# Autodesk Inventor assembly: 276-2194.html
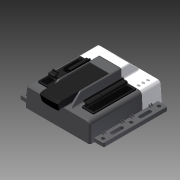
[picture p0: Inventor's stored thumbnail of the model, 180x180]
Saved by Autodesk Inventor 2013 (Build 170138000, 138)
## iProperties
Category: Logic
Company: Autodesk Inc.
Created: 2012-04-09
Part Number: 276-2194.html
Document SubType Name: Assembly
Designer: Autodesk Inc.
Catalog Web Link: http://www.vexrobotics.com/products/accessories/logic/276-2194.html#
Vendor: VEX
Mass: 136.985 g
Surface Area: 1281.69 cm^2
Volume: 120.224 cm^3
Author: Autodesk Inc.
## Documents named in this file (12)
- C:\Data Folder\VEX 2012\VEX KOP Uploads\2013\Imperial\Logic\VEX Cortex Microcontroller.iam
- C:\Data Folder\VEX 2012\VEX 2012 KOP\Imported Components\Cortex\276-2194-001 Rev2.ipt
- C:\Data Folder\VEX 2012\VEX 2012 KOP\Imported Components\Cortex\276-2194-PWM_LOCK_BUCKET.ipt
- C:\Data Folder\VEX 2012\VEX 2012 KOP\Imported Components\Cortex\276-2194-2_0_PCB_ASSY_REV2_ANY_ASM.iam
- C:\Data Folder\VEX 2012\VEX 2012 KOP\Imported Components\Cortex\276-2194-MOTOR_LOCK_BUCKET.ipt
- C:\Data Folder\VEX 2012\VEX 2012 KOP\Imported Components\Cortex\276-2194-LONG_LOCK_TAB.ipt
- C:\Data Folder\VEX 2012\VEX 2012 KOP\Imported Components\Cortex\276-2194-SWITCH_BUTTON.ipt
- C:\Data Folder\VEX 2012\VEX 2012 KOP\Imported Components\Cortex\276-2194-SMALL_LOCK_TAB.ipt
- C:\Data Folder\VEX 2012\VEX 2012 KOP\Imported Components\Cortex\276-2194-LIGHTPIPE.ipt
- C:\Data Folder\VEX 2012\VEX 2012 KOP\Imported Components\Cortex\276-2194-BOTTOM-CASE.ipt
- C:\Data Folder\VEX 2012\VEX 2012 KOP\Imported Components\Cortex\276-2194-SHORT_LOCK_TAB.ipt
- C:\Data Folder\VEX 2012\VEX 2012 KOP\VEX Updated Files\VEX KOP 2011\Imperial\Components\WIFI-KEY.ipt
## Components (13 placed, 11 different names)
1. 276-2194-001 Rev2:1 — Insert:1, Insert:2, Insert:3, Angle:1, Angle:2, Angle:3, Mate:6, Mate:7, Mate:8, Angle:4, Mate:11, Mate:12, Angle:5, Angle:6
2. 276-2194-PWM_LOCK_BUCKET:1
3. 276-2194-2_0_PCB_ASSY_REV2_ANY_ASM:1 [sub-assembly] — Mate:10, Angle:4, Mate:11, Mate:13, Mate:14
4. 276-2194-MOTOR_LOCK_BUCKET:1 — Flush:1, Mate:4
5. 276-2194-LONG_LOCK_TAB:1
6. 276-2194-SWITCH_BUTTON:1
7. 276-2194-SMALL_LOCK_TAB:1 — Flush:1, Mate:4
8. 276-2194-LIGHTPIPE:1 — Insert:2, Angle:2
9. 276-2194-BOTTOM-CASE:1 — Mate:6, Mate:7, Mate:8, Mate:10
10. 276-2194-SHORT_LOCK_TAB:1
11. 276-2194-LIGHTPIPE:2 — Insert:1, Angle:1
12. 276-2194-LIGHTPIPE:3 — Insert:3, Angle:3
13. WIFI-KEY:1 — Flush:2, Angle:6, Mate:13, Mate:14
## Relationships (20: Mate 9, Angle 6, Insert 3, Flush 2)
- Insert:1: 276-2194-001 Rev2:1 ↔ 276-2194-LIGHTPIPE:2
- Insert:2: 276-2194-001 Rev2:1 ↔ 276-2194-LIGHTPIPE:1
- Insert:3: 276-2194-001 Rev2:1 ↔ 276-2194-LIGHTPIPE:3
- Angle:1 (0 deg): 276-2194-001 Rev2:1 ↔ 276-2194-LIGHTPIPE:2
- Angle:2 (0 deg): 276-2194-001 Rev2:1 ↔ 276-2194-LIGHTPIPE:1
- Angle:3 (0 deg): 276-2194-001 Rev2:1 ↔ 276-2194-LIGHTPIPE:3
- Flush:1 (-4.9784 mm): 276-2194-MOTOR_LOCK_BUCKET:1 ↔ 276-2194-SMALL_LOCK_TAB:1
- Mate:4: 276-2194-MOTOR_LOCK_BUCKET:1 ↔ 276-2194-SMALL_LOCK_TAB:1
- Mate:6: 276-2194-001 Rev2:1 ↔ 276-2194-BOTTOM-CASE:1
- Mate:7: 276-2194-001 Rev2:1 ↔ 276-2194-BOTTOM-CASE:1
- Mate:8: 276-2194-001 Rev2:1 ↔ 276-2194-BOTTOM-CASE:1
- Mate:10: 276-2194-2_0_PCB_ASSY_REV2_ANY_ASM:1 ↔ 276-2194-BOTTOM-CASE:1
- Angle:4 (0 deg): 276-2194-001 Rev2:1 ↔ 276-2194-2_0_PCB_ASSY_REV2_ANY_ASM:1
- Mate:11: 276-2194-001 Rev2:1 ↔ 276-2194-2_0_PCB_ASSY_REV2_ANY_ASM:1
- Mate:12: 276-2194-001 Rev2:1
- Angle:5 (0 deg): 276-2194-001 Rev2:1
- Flush:2: WIFI-KEY:1
- Angle:6 (180 deg): 276-2194-001 Rev2:1 ↔ WIFI-KEY:1
- Mate:13: 276-2194-2_0_PCB_ASSY_REV2_ANY_ASM:1 ↔ WIFI-KEY:1
- Mate:14: 276-2194-2_0_PCB_ASSY_REV2_ANY_ASM:1 ↔ WIFI-KEY:1
